# Autodesk Inventor assembly: Assy
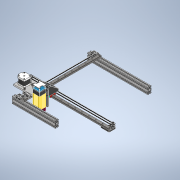
[picture p0: Inventor's stored thumbnail of the model, 180x180]
Saved by Autodesk Inventor 2022.2 (Build 262287010, 287A)
## iProperties
Created: 2022-05-03
Part Number: Assy
Document SubType Name: Assembly
Designer: MXBD
Author: MXBD
## Documents named in this file (7)
- D:\Laser_Engraver\CAD\Assembly\Assy.iam
- D:\Laser_Engraver\CAD\Assembly\03_XY_Assy.iam
- D:\Laser_Engraver\CAD\Parts\18_Aluprofil_350mm.ipt
- D:\Laser_Engraver\CAD\Parts\18_Aluprofil_250mm.ipt
- C:\Users\49152\Documents\Inventor\Content Center Files\R2022\de-DE\ISO 4762(2)\ISO 4762 - M3 x 10ISO.ipt
- D:\Laser_Engraver\CAD\Parts\19_Belt_holder.ipt
- D:\Laser_Engraver\CAD\Parts\20_Belt_450mm.ipt
## Components (8 placed, 6 different names)
1. 03_XY_Assy:1 [sub-assembly] — Passend:1, Passend:2, Fluchtend:1, Fluchtend:2, Fluchtend:3, Fluchtend:4, Passend:3, Passend:4, Passend:5, Passend:6, Passend:9, Passend:10
2. 18_Aluprofil_350mm:1 — Passend:2, Fluchtend:2, Fluchtend:4, Passend:8, Fluchtend:6
3. 18_Aluprofil_250mm:1 — Passend:1, Fluchtend:1, Fluchtend:3, Passend:7, Fluchtend:5
4. ISO 4762 M3 x 10:1 — Passend:3, Passend:6
5. ISO 4762 M3 x 10:2 — Passend:4, Passend:5
6. 19_Belt_holder:1 — Passend:8, Fluchtend:6, Passend:9, Passend:11, Passend:12, Passend:13
7. 19_Belt_holder:2 — Passend:7, Fluchtend:5, Passend:10
8. 20_Belt_450mm:1 — Passend:11, Passend:12, Passend:13
## Relationships (19: Mate 13, Flush 6)
- Passend:1 [Mate]: 03_XY_Assy:1 ↔ 18_Aluprofil_250mm:1
- Passend:2 [Mate]: 03_XY_Assy:1 ↔ 18_Aluprofil_350mm:1
- Fluchtend:1 [Flush] (-50 mm): 03_XY_Assy:1 ↔ 18_Aluprofil_250mm:1
- Fluchtend:2 [Flush] (-50 mm): 03_XY_Assy:1 ↔ 18_Aluprofil_350mm:1
- Fluchtend:3 [Flush] (-5 mm): 03_XY_Assy:1 ↔ 18_Aluprofil_250mm:1
- Fluchtend:4 [Flush] (-5 mm): 03_XY_Assy:1 ↔ 18_Aluprofil_350mm:1
- Passend:3 [Mate]: 03_XY_Assy:1 ↔ ISO 4762 M3 x 10:1
- Passend:4 [Mate]: 03_XY_Assy:1 ↔ ISO 4762 M3 x 10:2
- Passend:5 [Mate]: 03_XY_Assy:1 ↔ ISO 4762 M3 x 10:2
- Passend:6 [Mate]: 03_XY_Assy:1 ↔ ISO 4762 M3 x 10:1
- Passend:7 [Mate]: 18_Aluprofil_250mm:1 ↔ 19_Belt_holder:2
- Fluchtend:5 [Flush]: 18_Aluprofil_250mm:1 ↔ 19_Belt_holder:2
- Passend:8 [Mate]: 18_Aluprofil_350mm:1 ↔ 19_Belt_holder:1
- Fluchtend:6 [Flush]: 18_Aluprofil_350mm:1 ↔ 19_Belt_holder:1
- Passend:9 [Mate]: 03_XY_Assy:1 ↔ 19_Belt_holder:1
- Passend:10 [Mate]: 03_XY_Assy:1 ↔ 19_Belt_holder:2
- Passend:11 [Mate]: 19_Belt_holder:1 ↔ 20_Belt_450mm:1
- Passend:12 [Mate]: 19_Belt_holder:1 ↔ 20_Belt_450mm:1
- Passend:13 [Mate]: 19_Belt_holder:1 ↔ 20_Belt_450mm:1
